# Autodesk Inventor assembly: MIRarmアーム3
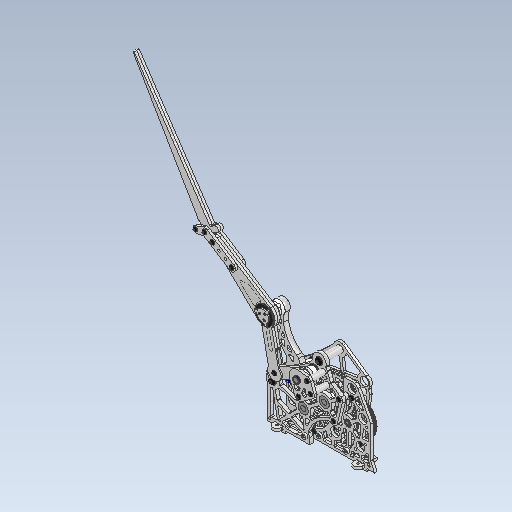
[picture p0: Inventor's stored thumbnail of the model, 512x512]
Saved by Autodesk Inventor 2020.3 (Build 243373000, 373)
## iProperties
Created: 2020-03-16
Part Number: MIRarmアーム3
Document SubType Name: Assembly
Designer: aoyama
Mass: 287.836 g
Surface Area: 1030.61 cm^2
Volume: 87.0511 cm^3
Density: 3.30652 g/cm^3
Author: aoyam
## Documents named in this file (51)
- C:\Users\aoyam\Desktop\SRDC_local\Inventor\二年機\Geminiβ\腕\MIR達\MIRarmアーム3.iam
- C:\Users\aoyam\Desktop\SRDC_local\Inventor\二年機\Geminiβ\腕\MIR達\MIRarmアーム用初段.iam
- C:\Users\aoyam\Desktop\SRDC_local\Inventor\二年機\Geminiβ\腕\MIR達\MIRarmアーム用2段.iam
- C:\Users\aoyam\Desktop\SRDC_local\Inventor\二年機\Geminiβ\腕\MIR達\MIRarmアーム用3段.iam
- C:\Users\aoyam\Desktop\SRDC_local\Inventor\二年機\Geminiβ\腕\MIR達\MIRarmモーターマウント改.ipt
- C:\Users\aoyam\Desktop\SRDC_local\Inventor\二年機\Geminiβ\腕\MIR達\MIRarmアームフレーム改二.ipt
- C:\Users\aoyam\Desktop\SRDC_local\Inventor\二年機\Geminiβ\汎用部品\MIR達\MIRarmベアリングHd6-D12-B4.ipt
- C:\Users\aoyam\Desktop\SRDC_local\Inventor\二年機\Geminiβ\汎用部品\MIR達\MIRarmベアリングd4D8B3F.ipt
- C:\Users\aoyam\Desktop\SRDC_local\Inventor\二年機\Geminiβ\汎用部品\MIR達\MIRarmスペーサー中空M6L3アルミ自作.ipt
- C:\Users\aoyam\Desktop\SRDC_local\Inventor\二年機\Geminiβ\腕\MIR達\MIRarmアームギアフレーム最内2.ipt
- C:\Users\aoyam\Desktop\SRDC_local\Inventor\二年機\Geminiβ\腕\MIR達\MIRarm駆動軸.ipt
- C:\Users\aoyam\Desktop\SRDC_local\Inventor\二年機\Geminiβ\汎用部品\MIR達\MIRarm平行ピンD6L28.ipt
- C:\Users\aoyam\Desktop\SRDC_local\Inventor\二年機\Geminiβ\汎用部品\MIR達\MIRarmワッシャD8d6m0.5.ipt
- C:\Users\aoyam\Desktop\SRDC_local\Inventor\二年機\Geminiβ\汎用部品\MIR達\MIRarmワッシャD7d4m0.5.ipt
- C:\Users\aoyam\Desktop\SRDC_local\Inventor\二年機\Geminiβ\汎用部品\MIR達\MIRarmスペーサーM6L5樹脂.ipt
- C:\Users\aoyam\Desktop\SRDC_local\Inventor\二年機\Geminiβ\汎用部品\MIR達\MIRarmスペーサーM6L8樹脂.ipt
- C:\Users\aoyam\Desktop\SRDC_local\Inventor\二年機\Geminiβ\汎用部品\MIR達\MIRarm平行ピンD4L18.ipt
- C:\Users\aoyam\Desktop\SRDC_local\Inventor\二年機\Geminiβ\汎用部品\MIR達\MIRarmスペーサーM3L12アルミ.ipt
- C:\Users\aoyam\Desktop\SRDC_local\Inventor\二年機\Geminiβ\汎用部品\MIR達\MIRarmスペーサーM3L6アルミ .ipt
- C:\Users\aoyam\Desktop\SRDC_local\Inventor\二年機\Geminiβ\腕\MIR達\MIRarmアーム揺動節test.ipt
- C:\Users\aoyam\Desktop\SRDC_local\Inventor\二年機\Geminiβ\腕\MIR達\MIRarmアーム中間節test.ipt
- C:\Users\aoyam\Desktop\SRDC_local\Inventor\二年機\Geminiβ\腕\MIR達\MIRarmアームカムAL.ipt
- C:\Users\aoyam\Desktop\SRDC_local\Inventor\二年機\Geminiβ\腕\MIR達\MIRarmアーム中間その弐.ipt
- C:\Users\aoyam\Desktop\SRDC_local\Inventor\二年機\Geminiβ\汎用部品\MIR達\MIRarmオイレスF外径16内径14L9.ipt
- C:\Users\aoyam\Desktop\SRDC_local\Inventor\二年機\Geminiβ\汎用部品\MIR達\MIRarmネジボタンM3L14.ipt
- C:\Users\aoyam\Desktop\SRDC_local\Inventor\二年機\Geminiβ\汎用部品\MIR達\MIRarmネジボタンM3L6.ipt
- C:\Users\aoyam\Desktop\SRDC_local\Inventor\二年機\Geminiβ\汎用部品\MIR達\MIRarmネジボタンM4L6.ipt
- C:\Users\aoyam\Desktop\SRDC_local\Inventor\二年機\Geminiβ\腕\MIR達\MIRarmアーム揺動節抑え.ipt
- C:\Users\aoyam\Desktop\SRDC_local\Inventor\二年機\Geminiβ\汎用部品\MIR達\MIRarmスペーサーM3L18アルミ.ipt
- C:\Users\aoyam\Desktop\SRDC_local\Inventor\二年機\Geminiβ\腕\MIR達\MIRarmアーム底板.ipt
- C:\Users\aoyam\Desktop\SRDC_local\Inventor\二年機\Geminiβ\腕\MIR達\MIRarmアーム先端.iam
- C:\Users\aoyam\Desktop\SRDC_local\Inventor\二年機\Geminiβ\汎用部品\MIR達\MIRarmオイレス外径8内径6L3.ipt
- C:\Users\aoyam\Desktop\SRDC_local\Inventor\二年機\Geminiβ\汎用部品\MIR達\MIRarmスペーサーM3L12樹脂.ipt
- C:\Users\aoyam\Desktop\SRDC_local\Inventor\二年機\Geminiβ\汎用部品\MIR達\MIRarmスペーサーM3L6樹脂.ipt
- C:\Users\aoyam\Desktop\SRDC_local\Inventor\二年機\Geminiβ\汎用部品\MIR達\MIRarmネジボタンM3L25.ipt
- C:\Users\aoyam\Desktop\SRDC_local\Inventor\二年機\Geminiβ\汎用部品\電子機器類\RDC506018A\RDC506018A.ipt
- C:\Users\aoyam\Desktop\SRDC_local\Inventor\二年機\Geminiβ\汎用部品\平行ピンD6L30Dcut.ipt
- C:\Users\aoyam\Desktop\SRDC_local\Inventor\二年機\Geminiβ\汎用部品\ネジボタンM2L6.ipt
- C:\Users\aoyam\Desktop\SRDC_local\Inventor\二年機\Geminiβ\汎用部品\平行ピンD6L28.ipt
- C:\Users\aoyam\Desktop\SRDC_local\Inventor\二年機\Geminiβ\腕\アームカムD15t4.ipt
- C:\Users\aoyam\Desktop\SRDC_local\Inventor\二年機\Geminiβ\腕\アームカムD14.ipt
- C:\Users\aoyam\Desktop\SRDC_local\Inventor\二年機\Geminiβ\腕\アームカムFD18t4.ipt
- C:\Users\aoyam\Desktop\SRDC_local\Inventor\二年機\Geminiβ\腕\アームカムD18.ipt
- C:\Users\aoyam\Desktop\SRDC_local\Inventor\二年機\Geminiβ\汎用部品\スペーサー中空M6L2.5樹脂自作.ipt
- C:\Users\aoyam\Desktop\SRDC_local\Inventor\二年機\Geminiβ\汎用部品\ワッシャD8d6m0.5.ipt
- C:\Users\aoyam\Desktop\SRDC_local\Inventor\二年機\Geminiβ\汎用部品\スペーサーM4L21アルミ.ipt
- C:\Users\aoyam\Desktop\SRDC_local\Inventor\二年機\Geminiβ\汎用部品\ネジアルミM3L6.ipt
- C:\Users\aoyam\Desktop\SRDC_local\Inventor\二年機\Geminiβ\汎用部品\ネジボタンM3L12.ipt
- C:\Users\aoyam\Desktop\SRDC_local\Inventor\二年機\Geminiβ\汎用部品\スペーサー中空M6L12樹脂.ipt
- C:\Users\aoyam\Desktop\SRDC_local\Inventor\二年機\Geminiβ\汎用部品\スペーサー中空M6L6樹脂.ipt
- C:\Users\aoyam\Desktop\SRDC_local\Inventor\二年機\Geminiβ\汎用部品\オイレスFd6D8L6.ipt
## Components (96 placed, 50 different names)
1. MIRarmアーム用初段:1 [sub-assembly] — メイト:4, 挿入:113
2. MIRarmアーム用2段:1 [sub-assembly] — メイト:4, メイト:21, メイト:6, メイト:27, 挿入:16, 挿入:151, 挿入:31
3. MIRarmアーム用3段:1 [sub-assembly] — メイト:21, メイト:6, メイト:28, 挿入:41
4. MIRarmモーターマウント改:1 — メイト:26, メイト:30, 挿入:47, 挿入:109, メイト:73, 挿入:165, 挿入:166, 挿入:120, 挿入:123, 挿入:138, 挿入:140, 挿入:141
5. MIRarmアームフレーム改二:1 — メイト:28, メイト:27, メイト:26, 挿入:13, 挿入:12, 挿入:14, 挿入:32, 挿入:46, 挿入:162, 挿入:135, メイト:74, 挿入:119, 挿入:122, 挿入:136, 挿入:137, メイト:29, 挿入:151
6. MIRarmベアリングHd6-D12-B4:1 — 挿入:13, 挿入:27
7. MIRarmベアリングd4D8B3F:1 — 挿入:12, 挿入:36, 挿入:42
8. MIRarmベアリングHd6-D12-B4:2 — 挿入:14, 挿入:28, 挿入:33
9. MIRarmスペーサー中空M6L3アルミ自作:1 — 挿入:16
10. MIRarmベアリングd4D8B3F:2 — 挿入:37, 挿入:120
11. MIRarmアームギアフレーム最内2:1 — メイト:30, 挿入:19, 挿入:20, 挿入:35, 挿入:123, メイト:32, 挿入:105, 挿入:107, 挿入:110, 挿入:126, 挿入:150, メイト:71, メイト:70, メイト:69, 挿入:143, 挿入:144, 挿入:145, メイト:72, 挿入:83, 挿入:84, 挿入:118, 挿入:121, 挿入:139, 挿入:145, 挿入:148, 挿入:150, 角度:2, 挿入:152
12. MIRarmベアリングHd6-D12-B4:3 — 挿入:19, メイト:54, 挿入:30
13. MIRarmベアリングHd6-D12-B4:4 — 挿入:20
14. MIRarm駆動軸:1 — 挿入:168, 挿入:167, 挿入:169, 挿入:109, 挿入:147, メイト:28
15. MIRarm平行ピンD6L28:1 — メイト:54, 挿入:27
16. MIRarm平行ピンD6L28:2 — 挿入:28
17. MIRarmワッシャD8d6m0.5:1 — 挿入:151
18. MIRarmワッシャD8d6m0.5:2 — 挿入:30, 挿入:39
19. MIRarmワッシャD8d6m0.5:3 — 挿入:31
20. MIRarmワッシャD8d6m0.5:4 — 挿入:32
21. MIRarmワッシャD8d6m0.5:5 — 挿入:33
22. MIRarmワッシャD8d6m0.5:6 — 挿入:35, 挿入:116
23. MIRarmワッシャD7d4m0.5:2 — 挿入:37, 挿入:114
24. MIRarmワッシャD7d4m0.5:3 — 挿入:36, 挿入:113
25. MIRarmスペーサーM6L5樹脂:1 — 挿入:39
26. MIRarmスペーサーM6L8樹脂:1 — 挿入:41
27. MIRarm平行ピンD4L18:1 — 挿入:42
28. MIRarmスペーサーM3L12アルミ:1 — 挿入:46
29. MIRarmスペーサーM3L6アルミ :1 — 挿入:123, 挿入:47
30. MIRarmアーム揺動節test:1 — メイト:32, 挿入:122, 挿入:142, 挿入:146
31. MIRarmアーム中間節test:1 — メイト:53, 挿入:120, 挿入:158, 挿入:124, 挿入:131
32. MIRarmアームカムAL:1 — 挿入:102, 挿入:103, 挿入:104, 挿入:105, 挿入:107
33. MIRarmアーム中間その弐:1 — 挿入:122, メイト:53, 挿入:120, 挿入:159, 挿入:98, 挿入:106
34. MIRarmオイレスF外径16内径14L9:1 — 挿入:102, 挿入:106, メイト:25, メイト:26, 挿入:111
35. MIRarmスペーサーM3L6アルミ :2 — 挿入:105
36. MIRarmネジボタンM3L14:1 — 挿入:107
37. MIRarmネジボタンM3L6:1 — 挿入:123
38. MIRarmネジボタンM3L6:2 — 挿入:109
39. MIRarmネジボタンM3L6:3 — 挿入:110
40. MIRarmネジボタンM3L6:4 — 挿入:122
41. MIRarmネジボタンM4L6:1 — 挿入:162
42. MIRarmネジボタンM4L6:2 — 挿入:126
43. MIRarmネジボタンM4L6:3 — 挿入:150
44. MIRarmネジボタンM4L6:4 — 挿入:135
45. MIRarmアーム揺動節抑え:1 — メイト:71, メイト:70, メイト:69, 挿入:140, 挿入:141, 挿入:142, 挿入:146, 挿入:147, 挿入:148
46. MIRarmスペーサーM3L18アルミ:1 — 挿入:140
47. MIRarmスペーサーM3L18アルミ:2 — 挿入:141, 挿入:148
48. MIRarmスペーサーM3L18アルミ:3 — 挿入:142
49. MIRarmネジボタンM3L6:11 — 挿入:143
50. MIRarmネジボタンM3L6:12 — 挿入:144
51. MIRarmネジボタンM3L6:13 — 挿入:145
52. MIRarmネジボタンM3L6:14 — 挿入:146
53. MIRarmネジボタンM3L6:15 — 挿入:147
54. MIRarmネジボタンM3L6:16 — 挿入:148
55. MIRarmアーム底板:1 — メイト:74, メイト:73, メイト:72
56. MIRarmアーム先端:1 [sub-assembly] — 挿入:98, 挿入:131, 挿入:132, 挿入:133, 挿入:134, 挿入:135
57. MIRarmオイレス外径8内径6L3:1 — 挿入:158
58. MIRarmネジボタンM3L6:17 — 挿入:159
59. MIRarmスペーサーM3L12樹脂:1 — 挿入:165
60. MIRarmスペーサーM3L12樹脂:2 — 挿入:166
61. MIRarmスペーサーM3L6樹脂:1 — 挿入:152
62. MIRarmネジボタンM3L25:1 — 挿入:168, 挿入:105
63. MIRarmネジボタンM3L25:2 — 挿入:167, 挿入:104
64. MIRarmネジボタンM3L25:3 — 挿入:169, 挿入:103, メイト:27
65. RDC506018A:1 — 挿入:82, 角度:1, メイト:30, 角度:2
66. 平行ピンD6L30Dcut:1 — 挿入:82, 角度:1, メイト:28, メイト:29
67. ネジボタンM2L6:1 — 挿入:83
68. ネジボタンM2L6:2 — 挿入:84
69. 平行ピンD6L28:1
70. アームカムD14:2 — 挿入:107, メイト:25, 挿入:108
71. アームカムD14:3 — 挿入:108, メイト:26
72. アームカムD15t4:1 — 挿入:109, メイト:27, 挿入:110
73. アームカムFD18t4:1 — 挿入:110, 挿入:111
74. アームカムD18:1 — 挿入:124
75. スペーサー中空M6L2.5樹脂自作:1 — 挿入:114
76. ワッシャD8d6m0.5:1 — 挿入:115, 挿入:116
77. ワッシャD8d6m0.5:2 — 挿入:115
78. スペーサーM4L21アルミ:1 — 挿入:119, 挿入:121
79. スペーサーM4L21アルミ:2 — 挿入:118
80. ネジアルミM3L6:1 — 挿入:137
81. ネジアルミM3L6:2 — 挿入:139
82. ネジアルミM3L6:3 — 挿入:141
83. ネジアルミM3L6:4 — 挿入:136
84. ネジアルミM3L6:5 — 挿入:138
85. ネジアルミM3L6:6 — 挿入:140
86. ネジボタンM3L12:1 — 挿入:132
87. ネジボタンM3L12:2 — 挿入:133
88. ネジボタンM3L12:3 — 挿入:134
89. ネジボタンM3L12:4 — 挿入:135
90. スペーサー中空M6L12樹脂:1 — 挿入:147, 挿入:149
91. スペーサー中空M6L6樹脂:1 — 挿入:144, 挿入:146
92. スペーサー中空M6L6樹脂:2 — 挿入:142, 挿入:143
93. オイレスFd6D8L6:1 — 挿入:143
94. オイレスFd6D8L6:2 — 挿入:144, 挿入:145
95. オイレスFd6D8L6:3 — 挿入:150, メイト:30
96. オイレスFd6D8L6:4 — 挿入:149, 挿入:151
## Relationships (119: Insert 95, Mate 22, Angle 2)
- メイト:4 [Mate] (0.5 mm): MIRarmアーム用初段:1 ↔ MIRarmアーム用2段:1
- メイト:21 [Mate] (0.5 mm): MIRarmアーム用2段:1 ↔ MIRarmアーム用3段:1
- メイト:6 [Mate] (0.5 mm): MIRarmアーム用2段:1 ↔ MIRarmアーム用3段:1
- メイト:28 [Mate]: MIRarmアーム用3段:1 ↔ MIRarmアームフレーム改二:1
- メイト:27 [Mate]: MIRarmアーム用2段:1 ↔ MIRarmアームフレーム改二:1
- メイト:26 [Mate]: MIRarmモーターマウント改:1 ↔ MIRarmアームフレーム改二:1
- 挿入:13 [Insert]: MIRarmアームフレーム改二:1 ↔ MIRarmベアリングHd6-D12-B4:1
- 挿入:12 [Insert]: MIRarmアームフレーム改二:1 ↔ MIRarmベアリングd4D8B3F:1
- 挿入:14 [Insert]: MIRarmアームフレーム改二:1 ↔ MIRarmベアリングHd6-D12-B4:2
- 挿入:16 [Insert] (0.5 mm): MIRarmアーム用2段:1 ↔ MIRarmスペーサー中空M6L3アルミ自作:1
- メイト:30 [Mate]: MIRarmモーターマウント改:1 ↔ MIRarmアームギアフレーム最内2:1
- 挿入:19 [Insert]: MIRarmアームギアフレーム最内2:1 ↔ MIRarmベアリングHd6-D12-B4:3
- 挿入:20 [Insert]: MIRarmアームギアフレーム最内2:1 ↔ MIRarmベアリングHd6-D12-B4:4
- メイト:54 [Mate]: MIRarmベアリングHd6-D12-B4:3 ↔ MIRarm平行ピンD6L28:1
- 挿入:27 [Insert]: MIRarmベアリングHd6-D12-B4:1 ↔ MIRarm平行ピンD6L28:1
- 挿入:28 [Insert]: MIRarmベアリングHd6-D12-B4:2 ↔ MIRarm平行ピンD6L28:2
- 挿入:151 [Insert]: MIRarmアーム用2段:1 ↔ MIRarmワッシャD8d6m0.5:1
- 挿入:30 [Insert]: MIRarmベアリングHd6-D12-B4:3 ↔ MIRarmワッシャD8d6m0.5:2
- 挿入:31 [Insert]: MIRarmアーム用2段:1 ↔ MIRarmワッシャD8d6m0.5:3
- 挿入:32 [Insert]: MIRarmアームフレーム改二:1 ↔ MIRarmワッシャD8d6m0.5:4
- 挿入:33 [Insert]: MIRarmベアリングHd6-D12-B4:2 ↔ MIRarmワッシャD8d6m0.5:5
- 挿入:35 [Insert]: MIRarmアームギアフレーム最内2:1 ↔ MIRarmワッシャD8d6m0.5:6
- 挿入:37 [Insert]: MIRarmベアリングd4D8B3F:2 ↔ MIRarmワッシャD7d4m0.5:2
- 挿入:36 [Insert]: MIRarmベアリングd4D8B3F:1 ↔ MIRarmワッシャD7d4m0.5:3
- 挿入:39 [Insert]: MIRarmワッシャD8d6m0.5:2 ↔ MIRarmスペーサーM6L5樹脂:1
- 挿入:41 [Insert]: MIRarmアーム用3段:1 ↔ MIRarmスペーサーM6L8樹脂:1
- 挿入:42 [Insert]: MIRarmベアリングd4D8B3F:1 ↔ MIRarm平行ピンD4L18:1
- 挿入:46 [Insert]: MIRarmアームフレーム改二:1 ↔ MIRarmスペーサーM3L12アルミ:1
- 挿入:123 [Insert]: MIRarmアームギアフレーム最内2:1 ↔ MIRarmスペーサーM3L6アルミ :1
- 挿入:47 [Insert]: MIRarmモーターマウント改:1 ↔ MIRarmスペーサーM3L6アルミ :1
- メイト:32 [Mate]: MIRarmアームギアフレーム最内2:1 ↔ MIRarmアーム揺動節test:1
- 挿入:122 [Insert]: MIRarmアーム揺動節test:1 ↔ MIRarmアーム中間その弐:1
- メイト:53 [Mate]: MIRarmアーム中間節test:1 ↔ MIRarmアーム中間その弐:1
- 挿入:120 [Insert]: MIRarmアーム中間節test:1 ↔ MIRarmアーム中間その弐:1
- 挿入:105 [Insert]: MIRarmアームギアフレーム最内2:1 ↔ MIRarmスペーサーM3L6アルミ :2
- 挿入:107 [Insert]: MIRarmアームギアフレーム最内2:1 ↔ MIRarmネジボタンM3L14:1
- 挿入:109 [Insert]: MIRarmモーターマウント改:1 ↔ MIRarmネジボタンM3L6:2
- 挿入:110 [Insert]: MIRarmアームギアフレーム最内2:1 ↔ MIRarmネジボタンM3L6:3
- 挿入:162 [Insert]: MIRarmアームフレーム改二:1 ↔ MIRarmネジボタンM4L6:1
- 挿入:126 [Insert]: MIRarmアームギアフレーム最内2:1 ↔ MIRarmネジボタンM4L6:2
- 挿入:150 [Insert]: MIRarmアームギアフレーム最内2:1 ↔ MIRarmネジボタンM4L6:3
- 挿入:135 [Insert]: MIRarmアームフレーム改二:1 ↔ MIRarmネジボタンM4L6:4
- メイト:71 [Mate]: MIRarmアームギアフレーム最内2:1 ↔ MIRarmアーム揺動節抑え:1
- メイト:70 [Mate]: MIRarmアームギアフレーム最内2:1 ↔ MIRarmアーム揺動節抑え:1
- メイト:69 [Mate]: MIRarmアームギアフレーム最内2:1 ↔ MIRarmアーム揺動節抑え:1
- 挿入:140 [Insert]: MIRarmアーム揺動節抑え:1 ↔ MIRarmスペーサーM3L18アルミ:1
- 挿入:141 [Insert]: MIRarmアーム揺動節抑え:1 ↔ MIRarmスペーサーM3L18アルミ:2
- 挿入:142 [Insert]: MIRarmアーム揺動節抑え:1 ↔ MIRarmスペーサーM3L18アルミ:3
- 挿入:143 [Insert]: MIRarmアームギアフレーム最内2:1 ↔ MIRarmネジボタンM3L6:11
- 挿入:144 [Insert]: MIRarmアームギアフレーム最内2:1 ↔ MIRarmネジボタンM3L6:12
- 挿入:145 [Insert]: MIRarmアームギアフレーム最内2:1 ↔ MIRarmネジボタンM3L6:13
- 挿入:146 [Insert]: MIRarmアーム揺動節抑え:1 ↔ MIRarmネジボタンM3L6:14
- 挿入:147 [Insert]: MIRarmアーム揺動節抑え:1 ↔ MIRarmネジボタンM3L6:15
- 挿入:148 [Insert]: MIRarmアーム揺動節抑え:1 ↔ MIRarmネジボタンM3L6:16
- メイト:74 [Mate]: MIRarmアームフレーム改二:1 ↔ MIRarmアーム底板:1
- メイト:73 [Mate]: MIRarmモーターマウント改:1 ↔ MIRarmアーム底板:1
- メイト:72 [Mate]: MIRarmアームギアフレーム最内2:1 ↔ MIRarmアーム底板:1
- 挿入:158 [Insert]: MIRarmアーム中間節test:1 ↔ MIRarmオイレス外径8内径6L3:1
- 挿入:159 [Insert]: MIRarmアーム中間その弐:1 ↔ MIRarmネジボタンM3L6:17
- 挿入:165 [Insert]: MIRarmモーターマウント改:1 ↔ MIRarmスペーサーM3L12樹脂:1
- 挿入:166 [Insert]: MIRarmモーターマウント改:1 ↔ MIRarmスペーサーM3L12樹脂:2
- 挿入:168 [Insert]: MIRarm駆動軸:1 ↔ MIRarmネジボタンM3L25:1
- 挿入:167 [Insert]: MIRarm駆動軸:1 ↔ MIRarmネジボタンM3L25:2
- 挿入:169 [Insert]: MIRarm駆動軸:1 ↔ MIRarmネジボタンM3L25:3
- 挿入:82 [Insert]: RDC506018A:1 ↔ 平行ピンD6L30Dcut:1
- 角度:1 [Angle] (180 deg): RDC506018A:1 ↔ 平行ピンD6L30Dcut:1
- 挿入:83 [Insert] (0.1 mm): MIRarmアームギアフレーム最内2:1 ↔ ネジボタンM2L6:1
- 挿入:84 [Insert] (0.1 mm): MIRarmアームギアフレーム最内2:1 ↔ ネジボタンM2L6:2
- 挿入:98 [Insert]: MIRarmアーム中間その弐:1 ↔ MIRarmアーム先端:1
- 挿入:102 [Insert]: MIRarmアームカムAL:1 ↔ MIRarmオイレスF外径16内径14L9:1
- 挿入:103 [Insert]: MIRarmアームカムAL:1 ↔ MIRarmネジボタンM3L25:3
- 挿入:104 [Insert]: MIRarmアームカムAL:1 ↔ MIRarmネジボタンM3L25:2
- 挿入:105 [Insert]: MIRarmアームカムAL:1 ↔ MIRarmネジボタンM3L25:1
- 挿入:106 [Insert]: MIRarmアーム中間その弐:1 ↔ MIRarmオイレスF外径16内径14L9:1
- 挿入:107 [Insert]: MIRarmアームカムAL:1 ↔ アームカムD14:2
- メイト:25 [Mate]: MIRarmオイレスF外径16内径14L9:1 ↔ アームカムD14:2
- 挿入:108 [Insert]: アームカムD14:2 ↔ アームカムD14:3
- メイト:26 [Mate]: MIRarmオイレスF外径16内径14L9:1 ↔ アームカムD14:3
- 挿入:109 [Insert]: MIRarm駆動軸:1 ↔ アームカムD15t4:1
- メイト:27 [Mate]: MIRarmネジボタンM3L25:3 ↔ アームカムD15t4:1
- 挿入:110 [Insert]: アームカムD15t4:1 ↔ アームカムFD18t4:1
- 挿入:111 [Insert]: MIRarmオイレスF外径16内径14L9:1 ↔ アームカムFD18t4:1
- 挿入:113 [Insert]: MIRarmアーム用初段:1 ↔ MIRarmワッシャD7d4m0.5:3
- 挿入:114 [Insert]: MIRarmワッシャD7d4m0.5:2 ↔ スペーサー中空M6L2.5樹脂自作:1
- 挿入:115 [Insert]: ワッシャD8d6m0.5:1 ↔ ワッシャD8d6m0.5:2
- 挿入:116 [Insert]: MIRarmワッシャD8d6m0.5:6 ↔ ワッシャD8d6m0.5:1
- 挿入:118 [Insert]: MIRarmアームギアフレーム最内2:1 ↔ スペーサーM4L21アルミ:2
- 挿入:119 [Insert]: MIRarmアームフレーム改二:1 ↔ スペーサーM4L21アルミ:1
- 挿入:120 [Insert]: MIRarmモーターマウント改:1 ↔ MIRarmベアリングd4D8B3F:2
- 挿入:121 [Insert]: MIRarmアームギアフレーム最内2:1 ↔ スペーサーM4L21アルミ:1
- 挿入:122 [Insert]: MIRarmアームフレーム改二:1 ↔ MIRarmネジボタンM3L6:4
- 挿入:123 [Insert]: MIRarmモーターマウント改:1 ↔ MIRarmネジボタンM3L6:1
- 挿入:124 [Insert]: MIRarmアーム中間節test:1 ↔ アームカムD18:1
- 挿入:131 [Insert]: MIRarmアーム中間節test:1 ↔ MIRarmアーム先端:1
- 挿入:132 [Insert]: MIRarmアーム先端:1 ↔ ネジボタンM3L12:1
- 挿入:133 [Insert]: MIRarmアーム先端:1 ↔ ネジボタンM3L12:2
- 挿入:134 [Insert]: MIRarmアーム先端:1 ↔ ネジボタンM3L12:3
- 挿入:135 [Insert]: MIRarmアーム先端:1 ↔ ネジボタンM3L12:4
- 挿入:136 [Insert]: MIRarmアームフレーム改二:1 ↔ ネジアルミM3L6:4
- 挿入:137 [Insert]: MIRarmアームフレーム改二:1 ↔ ネジアルミM3L6:1
- 挿入:138 [Insert]: MIRarmモーターマウント改:1 ↔ ネジアルミM3L6:5
- 挿入:139 [Insert]: MIRarmアームギアフレーム最内2:1 ↔ ネジアルミM3L6:2
- 挿入:140 [Insert]: MIRarmモーターマウント改:1 ↔ ネジアルミM3L6:6
- 挿入:141 [Insert]: MIRarmモーターマウント改:1 ↔ ネジアルミM3L6:3
- 挿入:142 [Insert]: MIRarmアーム揺動節test:1 ↔ スペーサー中空M6L6樹脂:2
- 挿入:143 [Insert]: スペーサー中空M6L6樹脂:2 ↔ オイレスFd6D8L6:1
- 挿入:144 [Insert]: スペーサー中空M6L6樹脂:1 ↔ オイレスFd6D8L6:2
- 挿入:145 [Insert]: MIRarmアームギアフレーム最内2:1 ↔ オイレスFd6D8L6:2
- 挿入:146 [Insert]: MIRarmアーム揺動節test:1 ↔ スペーサー中空M6L6樹脂:1
- 挿入:147 [Insert]: MIRarm駆動軸:1 ↔ スペーサー中空M6L12樹脂:1
- メイト:28 [Mate]: MIRarm駆動軸:1 ↔ 平行ピンD6L30Dcut:1
- メイト:29 [Mate]: MIRarmアームフレーム改二:1 ↔ 平行ピンD6L30Dcut:1
- 挿入:148 [Insert]: MIRarmアームギアフレーム最内2:1 ↔ MIRarmスペーサーM3L18アルミ:2
- 挿入:149 [Insert]: スペーサー中空M6L12樹脂:1 ↔ オイレスFd6D8L6:4
- 挿入:150 [Insert]: MIRarmアームギアフレーム最内2:1 ↔ オイレスFd6D8L6:3
- 挿入:151 [Insert]: MIRarmアームフレーム改二:1 ↔ オイレスFd6D8L6:4
- メイト:30 [Mate]: RDC506018A:1 ↔ オイレスFd6D8L6:3
- 角度:2 [Angle] (0 deg): MIRarmアームギアフレーム最内2:1 ↔ RDC506018A:1
- 挿入:152 [Insert]: MIRarmアームギアフレーム最内2:1 ↔ MIRarmスペーサーM3L6樹脂:1
